# Autodesk Inventor assembly: right triangle support
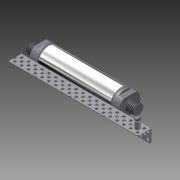
[picture p0: Inventor's stored thumbnail of the model, 180x180]
Saved by Autodesk Inventor 2014 SP1 (Build 180222100, 222)
## iProperties
Created: 2014-04-15
Part Number: right triangle support
Document SubType Name: Assembly
Designer: Ryan
Author: Ryan
## Documents named in this file (6)
- C:\Users\Ryan\Desktop\sw\toss up 5th A bot\tower\right triangle support.iam
- C:\Users\Ryan\Desktop\sw\lib\Aperture VEX CAD Library\Pnuematics\Reservoir.ipt
- C:\Users\Ryan\Desktop\sw\lib\Aperture VEX CAD Library\Metal\L Bar\2 x 19.ipt
- C:\Users\Ryan\Desktop\sw\lib\Aperture VEX CAD Library\Hardware\8-32\8-23_.750.ipt
- C:\Users\Ryan\Desktop\sw\lib\Aperture VEX CAD Library\Spacers\thin\SPACER-0320-0500.ipt
- C:\Users\Ryan\Desktop\sw\lib\Aperture VEX CAD Library\Hardware\8-32\8-32 nylock.ipt
## Components (5 placed, 5 different names)
1. Reservoir:1 — Tangent:1, Flush:1, Angle:1
2. 2 x 19:1 — Tangent:1, Flush:1, Angle:1, Mate:1, Mate:2, Mate:3, Mate:5
3. 8-23_.750:1 — Mate:1, Mate:2, Mate:3, Mate:4, Mate:6
4. SPACER-0320-0500:1 — Mate:4, Mate:5, Mate:7
5. 8-32 nylock:1 — Mate:6, Mate:7
## Relationships (10: Mate 7, Tangent 1, Flush 1, Angle 1)
- Tangent:1: Reservoir:1 ↔ 2 x 19:1
- Flush:1 (12.7 mm): Reservoir:1 ↔ 2 x 19:1
- Angle:1 (0 deg): Reservoir:1 ↔ 2 x 19:1
- Mate:1 (2.3114 mm): 2 x 19:1 ↔ 8-23_.750:1
- Mate:2: 2 x 19:1 ↔ 8-23_.750:1
- Mate:3 (2.3114 mm): 2 x 19:1 ↔ 8-23_.750:1
- Mate:4: 8-23_.750:1 ↔ SPACER-0320-0500:1
- Mate:5: 2 x 19:1 ↔ SPACER-0320-0500:1
- Mate:6: 8-23_.750:1 ↔ 8-32 nylock:1
- Mate:7 (1.1684 mm): SPACER-0320-0500:1 ↔ 8-32 nylock:1
## Named parameters: q = 2.3114 mm
